# Autodesk Inventor assembly: 麥克風組
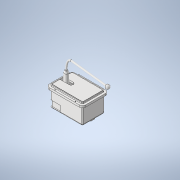
[picture p0: Inventor's stored thumbnail of the model, 180x180]
Saved by Autodesk Inventor 2021 (Build 250183000, 183)
## iProperties
Created: 2023-02-28
Part Number: 麥克風組
Document SubType Name: Assembly
Designer: brian
Author: brian
## Documents named in this file (4)
- C:\Users\brian\Desktop\自動主席台\麥克風組.iam
- C:\Users\brian\Desktop\自動主席台\麥克風崁座.ipt
- C:\Users\brian\Desktop\自動主席台\準確無線麥克風組.ipt
- C:\Users\brian\Desktop\自動主席台\新設計\麥克風蓋.ipt
## Components (3 placed, 3 different names)
1. 麥克風崁座:1 — 齊平:2, 齊平:3, 貼合:1, 齊平:4, 齊平:5
2. 準確無線麥克風組:1 — 齊平:2, 齊平:3, 貼合:1, 貼合:2
3. 麥克風蓋:1 — 貼合:2, 齊平:4, 齊平:5
## Relationships (6: Flush 4, Mate 2)
- 齊平:2 [Flush]: 麥克風崁座:1 ↔ 準確無線麥克風組:1
- 齊平:3 [Flush]: 麥克風崁座:1 ↔ 準確無線麥克風組:1
- 貼合:1 [Mate]: 麥克風崁座:1 ↔ 準確無線麥克風組:1
- 貼合:2 [Mate]: 準確無線麥克風組:1 ↔ 麥克風蓋:1
- 齊平:4 [Flush]: 麥克風崁座:1 ↔ 麥克風蓋:1
- 齊平:5 [Flush]: 麥克風崁座:1 ↔ 麥克風蓋:1
